# Autodesk Inventor assembly: cupula
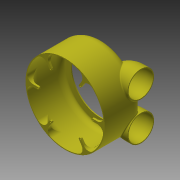
[picture p0: Inventor's stored thumbnail of the model, 180x180]
Saved by Autodesk Inventor 2015 (Build 190159000, 159)
## iProperties
Created: 2015-06-02
Part Number: cupula
Document SubType Name: Assembly
Designer: david_000
Author: david_000
## Documents named in this file (5)
- C:\Users\david_000\Desktop\minibot-code\mechanics\cupula.iam
- C:\Users\david_000\Desktop\minibot-code\mechanics\cupula_part_1.ipt
- C:\Users\david_000\Desktop\minibot-code\mechanics\cupula_part_2.ipt
- C:\Users\david_000\Desktop\minibot-code\mechanics\cupula_part_3.ipt
- C:\Users\david_000\Desktop\minibot-code\mechanics\cupula_part_4.ipt
## Components (4 placed, 4 different names)
1. cupula_part_1:1 — Coincidencia:1, Coincidencia:2, Coincidencia:3, Nivelación:1, Nivelación:3, Coincidencia:4, Coincidencia:5
2. cupula_part_2:1 — Coincidencia:2, Nivelación:3, Coincidencia:5, Coincidencia:6
3. cupula_part_3:1 — Coincidencia:1, Nivelación:1, Nivelación:2, Coincidencia:4
4. cupula_part_4:1 — Coincidencia:3, Nivelación:2, Coincidencia:6
## Relationships (9: Mate 6, Flush 3)
- Coincidencia:1 [Mate]: cupula_part_1:1 ↔ cupula_part_3:1
- Coincidencia:2 [Mate]: cupula_part_1:1 ↔ cupula_part_2:1
- Coincidencia:3 [Mate]: cupula_part_1:1 ↔ cupula_part_4:1
- Nivelación:1 [Flush]: cupula_part_1:1 ↔ cupula_part_3:1
- Nivelación:2 [Flush]: cupula_part_3:1 ↔ cupula_part_4:1
- Nivelación:3 [Flush]: cupula_part_1:1 ↔ cupula_part_2:1
- Coincidencia:4 [Mate]: cupula_part_1:1 ↔ cupula_part_3:1
- Coincidencia:5 [Mate]: cupula_part_1:1 ↔ cupula_part_2:1
- Coincidencia:6 [Mate]: cupula_part_2:1 ↔ cupula_part_4:1
